# Autodesk Inventor assembly: MGN7 Rail 150mm (3)
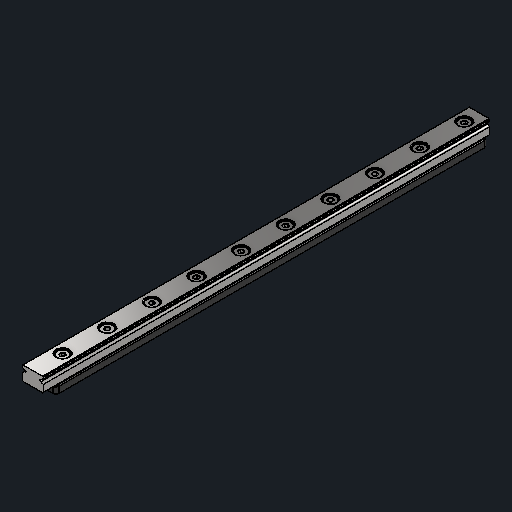
[picture p0: Inventor's stored thumbnail of the model, 512x512]
Saved by Autodesk Inventor 2026.1 (Build 301233020, 233B)
## iProperties
Created: 2025-05-09
Part Number: MGN7 Rail 150mm (3)
Document SubType Name: Assembly
Designer: AdminForWorker
Title: MGN7 150mm Rail
Author: AdminForWorker
## Documents named in this file (6)
- C:\Users\JoshuaEah\Documents\GitHub\Voron-0\CAD\Linear Rail\MGN7 Rail 150mm.iam
- MGN7 150mm Rail.iam
- C:\Users\JoshuaEah\Documents\GitHub\Voron-0\CAD\Hardware\M2x6 SHCS.ipt
- C:\Users\JoshuaEah\Documents\GitHub\Voron-0\CAD\Linear Rail\Parts\150 mm Rail.ipt
- C:\Users\JoshuaEah\Documents\GitHub\Voron-0\CAD\Linear Rail\Parts\M2 Hex Adapter.ipt
- C:\Users\JoshuaEah\Documents\GitHub\Voron-0\CAD\Hardware\M2 Hex Nut.ipt
## Components (22 placed, 4 different names)
1. 150mm Rail — Insert:1, Insert:2, Insert:3, Insert:4, Insert:5, Insert:6, Insert:7, Insert:8, Insert:9, Insert:10
2. M2x6 SHCS:1 — Insert:1
3. M2x6 SHCS:2 — Insert:6
4. M2x6 SHCS:3 — Insert:2
5. M2x6 SHCS:4 — Insert:9
6. M2x6 SHCS:5 — Insert:8
7. M2x6 SHCS:6 — Insert:4
8. M2x6 SHCS:7 — Insert:3
9. M2x6 SHCS:8 — Insert:7
10. M2x6 SHCS:9 — Insert:10
11. M2x6 SHCS:10 — Insert:5
12. M2 Hex Adapter:1
13. M2 Hex Nut:1
14. M2 Hex Nut:2
15. M2 Hex Nut:3
16. M2 Hex Nut:4
17. M2 Hex Nut:5
18. M2 Hex Nut:6
19. M2 Hex Nut:7
20. M2 Hex Nut:8
21. M2 Hex Nut:9
22. M2 Hex Nut:10
## Relationships (22: Insert 22)
- Insert:1: 150mm Rail ↔ M2x6 SHCS:1
- Insert:2: 150mm Rail ↔ M2x6 SHCS:3
- Insert:3: 150mm Rail ↔ M2x6 SHCS:7
- Insert:4: 150mm Rail ↔ M2x6 SHCS:6
- Insert:5: 150mm Rail ↔ M2x6 SHCS:10
- Insert:6: 150mm Rail ↔ M2x6 SHCS:2
- Insert:7: 150mm Rail ↔ M2x6 SHCS:8
- Insert:8: 150mm Rail ↔ M2x6 SHCS:5
- Insert:9: 150mm Rail ↔ M2x6 SHCS:4
- Insert:10: 150mm Rail ↔ M2x6 SHCS:9
- [Insert]: M2x6 SHCS:1 ↔ M2 Hex Nut:6
- [Insert]: M2x6 SHCS:9 ↔ M2 Hex Nut:3
- [Insert]: M2 Hex Adapter:1 ↔ M2 Hex Nut:6
- [Insert]: M2 Hex Adapter:1 ↔ M2 Hex Nut:4
- [Insert]: M2 Hex Adapter:1 ↔ M2 Hex Nut:7
- [Insert]: M2 Hex Adapter:1 ↔ M2 Hex Nut:10
- [Insert]: M2 Hex Adapter:1 ↔ M2 Hex Nut:5
- [Insert]: M2 Hex Adapter:1 ↔ M2 Hex Nut:9
- [Insert]: M2 Hex Adapter:1 ↔ M2 Hex Nut:2
- [Insert]: M2 Hex Adapter:1 ↔ M2 Hex Nut:8
- [Insert]: M2 Hex Adapter:1 ↔ M2 Hex Nut:1
- [Insert]: M2 Hex Adapter:1 ↔ M2 Hex Nut:3
